# Autodesk Inventor assembly: 6whalfdt_MIR
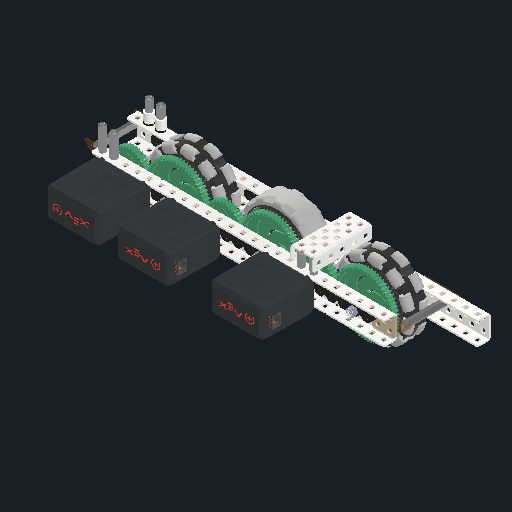
[picture p0: Inventor's stored thumbnail of the model, 512x512]
Saved by Autodesk Inventor 2024 (Build 280153000, 153)
## iProperties
Created: 2023-08-12
Part Number: 6whalfdt_MIR
Document SubType Name: Assembly
Designer: macbook
Author: macbook
## Documents named in this file (16)
- \\Mac\Home\Desktop\code\1599V-VRC\Cad\Assembly\v2\6whalfdt_MIR.iam
- \\Mac\Home\Desktop\code\1599V-VRC\Cad\Structure\C Channel\Aluminum 1x2x1\Alu C 1x2x1x25_MIR5.ipt
- \\Mac\Home\Desktop\code\1599V-VRC\Cad\Assembly\v2\omniwheel_MIR.iam
- \\Mac\Home\Desktop\code\1599V-VRC\Cad\Assembly\v2\gear_MIR.iam
- \\Mac\Home\Desktop\code\1599V-VRC\Cad\Assembly\v2\tractionwheel_MIR.iam
- \\Mac\Home\Desktop\code\1599V-VRC\Cad\Assembly\v2\sled-old_MIR.ipt
- \\Mac\Home\Desktop\code\1599V-VRC\Cad\Structure\Standoff\Standoff 2.00.ipt
- \\Mac\Home\Desktop\code\1599V-VRC\Cad\Structure\Standoff.ipt
- \\Mac\Home\Desktop\code\1599V-VRC\Cad\Structure\Standoff\Standoff .75.ipt
- \\Mac\Home\Desktop\code\1599V-VRC\Cad\Structure\C Channel\Aluminum 1x2x1\Alu C 1x2x1x5_MIR5.ipt
- \\Mac\Home\Desktop\code\1599V-VRC\Cad\Structure\Standoff\Standoff 1.00.ipt
- \\Mac\Home\Desktop\code\1599V-VRC\Cad\Structure\Standoff\Standoff .50.ipt
- \\Mac\Home\Desktop\code\1599V-VRC\Cad\Motion\Spacers\Spacer Nylon .313 OD\NSpacer .313 OD x .375.ipt
- \\Mac\Home\Desktop\code\1599V-VRC\Cad\Motion\Spacers\Spacer Nylon .313 OD.ipt
- \\Mac\Home\Desktop\code\1599V-VRC\Cad\Motion\Spacers\Spacer Nylon Click On\Nspacer Click On x .0625.ipt
- \\Mac\Home\Desktop\code\1599V-VRC\Cad\Motion\Spacers\Spacer Nylon Click On.ipt
## Components (27 placed, 12 different names)
1. Alu C 1x2x1x25_MIR5:1 — Insert:62, Insert:61, Insert:63, Insert:59, Insert:60, Insert:52, Insert:102, Insert:101, Insert:112, Insert:111, Insert:116, Insert:117, Insert:119, Insert:120
2. Alu C 1x2x1x25_MIR5:2 — Insert:105, Insert:54, Insert:103, Insert:58, Insert:60, Insert:52, Insert:108, Insert:80, Insert:104, Insert:55, Insert:107, Insert:106, Insert:110, Insert:109, Insert:114, Insert:115, Insert:124, Insert:125
3. omniwheel_MIR:1 [sub-assembly] — Insert:103, Insert:58
4. gear_MIR:1 [sub-assembly] — Insert:63, Insert:59
5. tractionwheel_MIR:1 [sub-assembly] — Insert:104, Insert:55
6. gear_MIR:2 [sub-assembly] — Insert:62, Insert:61
7. omniwheel_MIR:2 [sub-assembly] — Insert:105, Insert:54
8. gear_MIR:3 [sub-assembly] — Insert:107, Insert:106
9. sled-old_MIR:1 — Insert:108, Insert:80, Insert:100
10. sled-old_MIR:2 — Insert:102, Insert:101
11. Standoff 2.00:1 — Insert:100
12. sled-old_MIR:3 — Insert:110, Insert:109, Insert:113
13. sled-old_MIR:4 — Insert:112, Insert:111
14. Standoff 2.00:2 — Insert:113
15. Standoff .75:3 — Insert:114
16. Standoff .75:4 — Insert:115, Insert:118
17. Standoff .75:5 — Insert:116
18. Standoff .75:6 — Insert:117
19. Alu C 1x2x1x5_MIR5:1 — Insert:118
20. Standoff 1.00:7 — Insert:119
21. Standoff 1.00:8 — Insert:120
22. Standoff .50:9 — Insert:124, Insert:127
23. NSpacer .313 OD x .375:1 — Insert:123, Insert:128
24. Nspacer Click On x .0625:1 — Insert:123
25. Standoff .50:10 — Insert:128, Insert:125
26. NSpacer .313 OD x .375:2 — Insert:127, Insert:126
27. Nspacer Click On x .0625:2 — Insert:126
## Relationships (37: Insert 37)
- Insert:62: Alu C 1x2x1x25_MIR5:1 ↔ gear_MIR:2
- Insert:61: Alu C 1x2x1x25_MIR5:1 ↔ gear_MIR:2
- Insert:63: Alu C 1x2x1x25_MIR5:1 ↔ gear_MIR:1
- Insert:59: Alu C 1x2x1x25_MIR5:1 ↔ gear_MIR:1
- Insert:105: Alu C 1x2x1x25_MIR5:2 ↔ omniwheel_MIR:2
- Insert:54: Alu C 1x2x1x25_MIR5:2 ↔ omniwheel_MIR:2
- Insert:103: Alu C 1x2x1x25_MIR5:2 ↔ omniwheel_MIR:1
- Insert:58: Alu C 1x2x1x25_MIR5:2 ↔ omniwheel_MIR:1
- Insert:60 (49.2125 mm): Alu C 1x2x1x25_MIR5:1 ↔ Alu C 1x2x1x25_MIR5:2
- Insert:52 (49.2125 mm): Alu C 1x2x1x25_MIR5:1 ↔ Alu C 1x2x1x25_MIR5:2
- Insert:108: Alu C 1x2x1x25_MIR5:2 ↔ sled-old_MIR:1
- Insert:80: Alu C 1x2x1x25_MIR5:2 ↔ sled-old_MIR:1
- Insert:102: Alu C 1x2x1x25_MIR5:1 ↔ sled-old_MIR:2
- Insert:101: Alu C 1x2x1x25_MIR5:1 ↔ sled-old_MIR:2
- Insert:100: sled-old_MIR:1 ↔ Standoff 2.00:1
- Insert:104: Alu C 1x2x1x25_MIR5:2 ↔ tractionwheel_MIR:1
- Insert:55: Alu C 1x2x1x25_MIR5:2 ↔ tractionwheel_MIR:1
- Insert:107: Alu C 1x2x1x25_MIR5:2 ↔ gear_MIR:3
- Insert:106: Alu C 1x2x1x25_MIR5:2 ↔ gear_MIR:3
- Insert:110: Alu C 1x2x1x25_MIR5:2 ↔ sled-old_MIR:3
- Insert:109: Alu C 1x2x1x25_MIR5:2 ↔ sled-old_MIR:3
- Insert:112: Alu C 1x2x1x25_MIR5:1 ↔ sled-old_MIR:4
- Insert:111: Alu C 1x2x1x25_MIR5:1 ↔ sled-old_MIR:4
- Insert:113: sled-old_MIR:3 ↔ Standoff 2.00:2
- Insert:114: Alu C 1x2x1x25_MIR5:2 ↔ Standoff .75:3
- Insert:115: Alu C 1x2x1x25_MIR5:2 ↔ Standoff .75:4
- Insert:116: Alu C 1x2x1x25_MIR5:1 ↔ Standoff .75:5
- Insert:117: Alu C 1x2x1x25_MIR5:1 ↔ Standoff .75:6
- Insert:118: Standoff .75:4 ↔ Alu C 1x2x1x5_MIR5:1
- Insert:119: Alu C 1x2x1x25_MIR5:1 ↔ Standoff 1.00:7
- Insert:120: Alu C 1x2x1x25_MIR5:1 ↔ Standoff 1.00:8
- Insert:124 (12.7 mm): Alu C 1x2x1x25_MIR5:2 ↔ Standoff .50:9
- Insert:123: NSpacer .313 OD x .375:1 ↔ Nspacer Click On x .0625:1
- Insert:128: NSpacer .313 OD x .375:1 ↔ Standoff .50:10
- Insert:125 (12.7 mm): Alu C 1x2x1x25_MIR5:2 ↔ Standoff .50:10
- Insert:127: Standoff .50:9 ↔ NSpacer .313 OD x .375:2
- Insert:126: NSpacer .313 OD x .375:2 ↔ Nspacer Click On x .0625:2
